# Autodesk Inventor assembly: X Rail assy
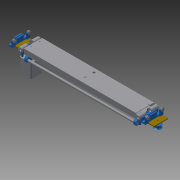
[picture p0: Inventor's stored thumbnail of the model, 180x180]
Saved by Autodesk Inventor 2013 SP2 (Build 170200200, 200)
## iProperties
Created: 2017-01-25
Part Number: X Rail assy
Document SubType Name: Assembly
Designer: Herman de Vries
Mass: 268.721 g
Surface Area: 1324.16 cm^2
Volume: 268.721 cm^3
Density: 1 g/cm^3
Author: Herman de Vries
## Documents named in this file (18)
- C:\Users\hdv\Dropbox\Projects\Inventor\PaintBot_3\X Rail assy.iam
- C:\Users\hdv\Dropbox\Projects\Inventor\PaintBot_3\X Rail.ipt
- C:\Users\hdv\Dropbox\Projects\Inventor\PaintBot_3\NEMA42.ipt
- C:\Users\hdv\Dropbox\Projects\Inventor\PaintBot_3\gear belt.ipt
- C:\Users\hdv\Dropbox\Projects\Inventor\PaintBot_3\Pully25mmx12mm.iam
- C:\Users\hdv\Dropbox\Projects\Inventor\PaintBot_3\spacer 6mmx10_5mm.ipt
- C:\Users\hdv\Dropbox\Projects\Inventor\PaintBot_3\spacer top 6mm.ipt
- C:\Users\hdv\Dropbox\Projects\Inventor\PaintBot_3\spacer stepperM.ipt
- C:\Users\hdv\Dropbox\Projects\Inventor\PaintBot_3\spacer stepperM n rail.ipt
- C:\Users\hdv\Dropbox\Projects\Inventor\PaintBot_3\x axis 8mm rod.ipt
- C:\Users\hdv\Dropbox\Projects\Inventor\PaintBot_3\Linear bearing 8mm.ipt
- C:\Users\hdv\Dropbox\Projects\Inventor\PaintBot_3\GT2 grip v2.ipt
- C:\Users\hdv\Dropbox\Projects\Inventor\PaintBot_3\bearing V groove 12mm.ipt
- C:\Users\hdv\Dropbox\Projects\Inventor\PaintBot_3\Linear bearing 8mm clamp.ipt
- C:\Users\hdv\Dropbox\Projects\Inventor\parts\P-BD000035 - Screw M3x10mm Hex Socket Head Cap SS ISO4762.ipt
- C:\Users\hdv\Dropbox\Projects\Inventor\parts\P-BD000005 - Screw M3x8mm Hex Socket Head Cap SS ISO4762.ipt
- C:\Users\hdv\Dropbox\Projects\Inventor\parts\P-BB000001 - Nut M3 Nyloc SS ISO7040.ipt
- C:\Users\hdv\Dropbox\Projects\Inventor\PaintBot_3\X Rail square.ipt
## Components (39 placed, 17 different names)
1. X Rail:1 — Mate:14, Insert:33, Insert:40, Insert:41, Insert:44, Insert:45, Mate:23, Flush:26, Mate:26, Flush:29, Flush:33, Insert:54, Insert:55, Mate:30, Flush:37, Mate:32, Mate:34, Flush:38, Flush:39, Flush:40, Flush:41, Insert:70, Insert:71, Insert:72, Insert:73
2. NEMA42:1 — Mate:20, Insert:42, Insert:43, Mate:29
3. gear belt:1 — Mate:20, Mate:29
4. Pully25mmx12mm:1 [sub-assembly] — Insert:19, Insert:20
5. spacer 6mmx10_5mm:1 — Insert:19, Insert:33
6. spacer top 6mm:1 — Insert:20
7. spacer stepperM:2 — Insert:42, Insert:44
8. spacer stepperM:3 — Insert:43, Insert:45
9. spacer stepperM n rail:1 — Insert:38, Insert:39, Insert:40, Insert:41
10. spacer stepperM n rail:2 — Mate:14, Insert:24, Insert:25
11. x axis 8mm rod:1 — Insert:24, Insert:39
12. x axis 8mm rod:2 — Insert:25, Insert:38
13. Linear bearing 8mm:1 — Mate:27, Flush:30
14. Linear bearing 8mm:2 — Mate:25, Flush:27
15. Linear bearing 8mm:3 — Mate:24, Flush:28
16. bearing V groove 12mm:1 — Insert:63, Insert:65
17. bearing V groove 12mm:2 — Insert:62, Insert:64
18. bearing V groove 12mm:3 — Insert:66, Insert:68
19. bearing V groove 12mm:4 — Insert:67, Insert:69
20. Linear bearing 8mm clamp:1 — Mate:23, Flush:26, Mate:24, Mate:25, Flush:27, Flush:28, Flush:33, Insert:46, Insert:47, Mate:31, Flush:36
21. Linear bearing 8mm clamp:2 — Mate:26, Flush:29, Mate:27, Flush:30, Mate:28, Flush:31, Insert:50, Insert:51, Flush:40
22. Linear bearing 8mm:4 — Mate:28, Flush:31
23. P-BD000035 - Screw M3x10mm Hex Socket Head Cap SS ISO4762:1 — Insert:46
24. P-BD000035 - Screw M3x10mm Hex Socket Head Cap SS ISO4762:2 — Insert:47
25. P-BD000035 - Screw M3x10mm Hex Socket Head Cap SS ISO4762:3 — Insert:50
26. P-BD000035 - Screw M3x10mm Hex Socket Head Cap SS ISO4762:4 — Insert:51
27. P-BD000005 - Screw M3x8mm Hex Socket Head Cap SS ISO4762:1 — Insert:72
28. P-BD000005 - Screw M3x8mm Hex Socket Head Cap SS ISO4762:2 — Insert:73
29. P-BD000005 - Screw M3x8mm Hex Socket Head Cap SS ISO4762:3 — Insert:71
30. P-BD000005 - Screw M3x8mm Hex Socket Head Cap SS ISO4762:4 — Insert:70
31. P-BB000001 - Nut M3 Nyloc SS ISO7040:1 — Insert:55
32. P-BB000001 - Nut M3 Nyloc SS ISO7040:2 — Insert:54
33. X Rail square:1 — Mate:30, Mate:31, Flush:36
34. P-BD000035 - Screw M3x10mm Hex Socket Head Cap SS ISO4762:5 — Insert:62
35. P-BD000035 - Screw M3x10mm Hex Socket Head Cap SS ISO4762:6 — Insert:63
36. P-BD000035 - Screw M3x10mm Hex Socket Head Cap SS ISO4762:7 — Insert:68
37. P-BD000035 - Screw M3x10mm Hex Socket Head Cap SS ISO4762:8 — Insert:69
38. GT2 grip v2:3 — Flush:37, Mate:32, Flush:39, Insert:66, Insert:67
39. GT2 grip v2:4 — Mate:34, Flush:38, Flush:41, Insert:64, Insert:65
## Relationships (57: Insert 31, Mate 13, Flush 13)
- Insert:19: Pully25mmx12mm:1 ↔ spacer 6mmx10_5mm:1
- Insert:20: Pully25mmx12mm:1 ↔ spacer top 6mm:1
- Mate:14: X Rail:1 ↔ spacer stepperM n rail:2
- Insert:24: spacer stepperM n rail:2 ↔ x axis 8mm rod:1
- Insert:25: spacer stepperM n rail:2 ↔ x axis 8mm rod:2
- Mate:20: NEMA42:1 ↔ gear belt:1
- Insert:33: X Rail:1 ↔ spacer 6mmx10_5mm:1
- Insert:38: spacer stepperM n rail:1 ↔ x axis 8mm rod:2
- Insert:39: spacer stepperM n rail:1 ↔ x axis 8mm rod:1
- Insert:40: X Rail:1 ↔ spacer stepperM n rail:1
- Insert:41: X Rail:1 ↔ spacer stepperM n rail:1
- Insert:42: NEMA42:1 ↔ spacer stepperM:2
- Insert:43: NEMA42:1 ↔ spacer stepperM:3
- Insert:44: X Rail:1 ↔ spacer stepperM:2
- Insert:45: X Rail:1 ↔ spacer stepperM:3
- Mate:23: X Rail:1 ↔ Linear bearing 8mm clamp:1
- Flush:26 (-10 mm): X Rail:1 ↔ Linear bearing 8mm clamp:1
- Mate:24: Linear bearing 8mm:3 ↔ Linear bearing 8mm clamp:1
- Mate:25: Linear bearing 8mm:2 ↔ Linear bearing 8mm clamp:1
- Flush:27: Linear bearing 8mm:2 ↔ Linear bearing 8mm clamp:1
- Flush:28: Linear bearing 8mm:3 ↔ Linear bearing 8mm clamp:1
- Mate:26: X Rail:1 ↔ Linear bearing 8mm clamp:2
- Flush:29 (-10 mm): X Rail:1 ↔ Linear bearing 8mm clamp:2
- Mate:27: Linear bearing 8mm:1 ↔ Linear bearing 8mm clamp:2
- Flush:30: Linear bearing 8mm:1 ↔ Linear bearing 8mm clamp:2
- Mate:28: Linear bearing 8mm clamp:2 ↔ Linear bearing 8mm:4
- Flush:31: Linear bearing 8mm clamp:2 ↔ Linear bearing 8mm:4
- Flush:33 (35 mm): X Rail:1 ↔ Linear bearing 8mm clamp:1
- Mate:29 (5 mm): NEMA42:1 ↔ gear belt:1
- Insert:46: Linear bearing 8mm clamp:1 ↔ P-BD000035 - Screw M3x10mm Hex Socket Head Cap SS ISO4762:1
- Insert:47: Linear bearing 8mm clamp:1 ↔ P-BD000035 - Screw M3x10mm Hex Socket Head Cap SS ISO4762:2
- Insert:50: Linear bearing 8mm clamp:2 ↔ P-BD000035 - Screw M3x10mm Hex Socket Head Cap SS ISO4762:3
- Insert:51: Linear bearing 8mm clamp:2 ↔ P-BD000035 - Screw M3x10mm Hex Socket Head Cap SS ISO4762:4
- Insert:54: X Rail:1 ↔ P-BB000001 - Nut M3 Nyloc SS ISO7040:2
- Insert:55: X Rail:1 ↔ P-BB000001 - Nut M3 Nyloc SS ISO7040:1
- Mate:30: X Rail:1 ↔ X Rail square:1
- Mate:31: Linear bearing 8mm clamp:1 ↔ X Rail square:1
- Flush:36: Linear bearing 8mm clamp:1 ↔ X Rail square:1
- Insert:62: bearing V groove 12mm:2 ↔ P-BD000035 - Screw M3x10mm Hex Socket Head Cap SS ISO4762:5
- Insert:63: bearing V groove 12mm:1 ↔ P-BD000035 - Screw M3x10mm Hex Socket Head Cap SS ISO4762:6
- Flush:37 (22 mm): X Rail:1 ↔ GT2 grip v2:3
- Mate:32: X Rail:1 ↔ GT2 grip v2:3
- Mate:34: X Rail:1 ↔ GT2 grip v2:4
- Flush:38 (12 mm): X Rail:1 ↔ GT2 grip v2:4
- Flush:39 (-12 mm): X Rail:1 ↔ GT2 grip v2:3
- Flush:40 (35 mm): X Rail:1 ↔ Linear bearing 8mm clamp:2
- Flush:41 (-2 mm): X Rail:1 ↔ GT2 grip v2:4
- Insert:64: bearing V groove 12mm:2 ↔ GT2 grip v2:4
- Insert:65: bearing V groove 12mm:1 ↔ GT2 grip v2:4
- Insert:66: bearing V groove 12mm:3 ↔ GT2 grip v2:3
- Insert:67: bearing V groove 12mm:4 ↔ GT2 grip v2:3
- Insert:68: bearing V groove 12mm:3 ↔ P-BD000035 - Screw M3x10mm Hex Socket Head Cap SS ISO4762:7
- Insert:69: bearing V groove 12mm:4 ↔ P-BD000035 - Screw M3x10mm Hex Socket Head Cap SS ISO4762:8
- Insert:70: X Rail:1 ↔ P-BD000005 - Screw M3x8mm Hex Socket Head Cap SS ISO4762:4
- Insert:71: X Rail:1 ↔ P-BD000005 - Screw M3x8mm Hex Socket Head Cap SS ISO4762:3
- Insert:72: X Rail:1 ↔ P-BD000005 - Screw M3x8mm Hex Socket Head Cap SS ISO4762:1
- Insert:73: X Rail:1 ↔ P-BD000005 - Screw M3x8mm Hex Socket Head Cap SS ISO4762:2
